# Autodesk Inventor assembly: plate_1set
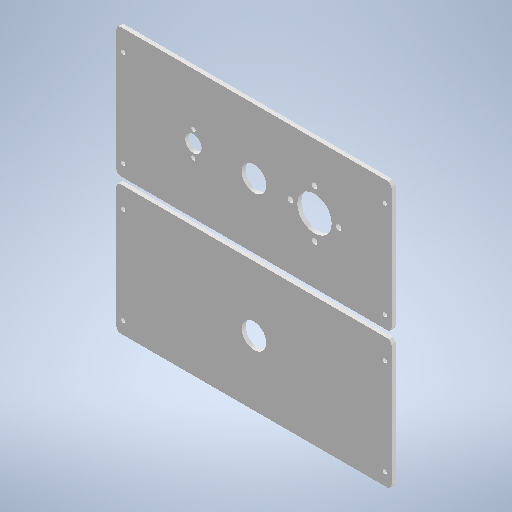
[picture p0: Inventor's stored thumbnail of the model, 512x512]
Saved by Autodesk Inventor 2025.1 (Build 291241000, 241)
## iProperties
Created: 2024-10-17
Part Number: plate_1set
Document SubType Name: Assembly
Designer: yuki0520
Author: yuki0520
## Documents named in this file (3)
- C:\Users\yuki0520\OneDrive\ドキュメント\Inventor\2025_nhk\tanaka\nageru\cnc\plate_1set.iam
- C:\Users\yuki0520\OneDrive\ドキュメント\Inventor\2025_nhk\tanaka\nageru\pakuriz\canon_plate.ipt
- C:\Users\yuki0520\OneDrive\ドキュメント\Inventor\2025_nhk\tanaka\nageru\pakuriz\canon_plate_motor.ipt
## Components (2 placed, 2 different names)
1. canon_plate:1 — フラッシュ:1, フラッシュ:2, メイト:1
2. canon_plate_motor:1 — フラッシュ:1, フラッシュ:2, メイト:1
## Relationships (3: Flush 2, Mate 1)
- フラッシュ:1 [Flush]: canon_plate:1 ↔ canon_plate_motor:1
- フラッシュ:2 [Flush]: canon_plate:1 ↔ canon_plate_motor:1
- メイト:1 [Mate] (5 mm): canon_plate:1 ↔ canon_plate_motor:1
